# Autodesk Inventor assembly: Heatsink+fan RPi-5
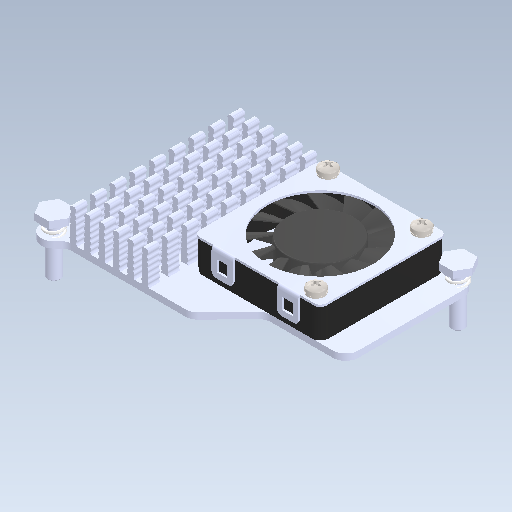
[picture p0: Inventor's stored thumbnail of the model, 512x512]
Saved by Autodesk Inventor 2021 (Build 250183000, 183)
## iProperties
Created: 2023-11-12
Part Number: Heatsink+fan RPi-5
Description: STEP AP214
Document SubType Name: Assembly
Designer: 22liatho
Sending System: SolidWorks 2021
Preprocessor: SwSTEP 2.0
Title: Heatsink+fan RPi-5.STEP
Revision Number: ANY
## Documents named in this file (7)
- C:\Users\22liatho\OneDrive - ABB Gymnasiet\Årskurs 3\Profil\Gymnasiearbete\GyArb Hållare CAD\CAD-filer\Raspberry_Pi_Heatsink+fan.iam
- C:\Users\22liatho\OneDrive - ABB Gymnasiet\Årskurs 3\Profil\Gymnasiearbete\GyArb Hållare CAD\CAD-filer\Heatsink-fan-base_RPi5.ipt
- C:\Users\22liatho\OneDrive - ABB Gymnasiet\Årskurs 3\Profil\Gymnasiearbete\GyArb Hållare CAD\CAD-filer\Fan_Assembly.iam
- C:\Users\22liatho\OneDrive - ABB Gymnasiet\Årskurs 3\Profil\Gymnasiearbete\GyArb Hållare CAD\CAD-filer\Fan_Cover.ipt
- C:\Users\22liatho\OneDrive - ABB Gymnasiet\Årskurs 3\Profil\Gymnasiearbete\GyArb Hållare CAD\CAD-filer\Spring-bolt_M2,5.iam
- C:\Users\22liatho\OneDrive - ABB Gymnasiet\Årskurs 3\Profil\Gymnasiearbete\GyArb Hållare CAD\CAD-filer\pan_head_cross_recess_screw_din_DIN_EN_ISO_7045_-_M2_x_10_-_Z_-_10N.ipt
- C:\Users\22liatho\OneDrive - ABB Gymnasiet\Årskurs 3\Profil\Gymnasiearbete\GyArb Hållare CAD\CAD-filer\plain_washer_small_grade_a_din_Washer_DIN_433_-_2.ipt
## Components (11 placed, 11 different names)
1. Heatsink-fan-base_RPi5_1 — Mate:1, Mate:2, Mate:3, Mate:4
2. final_assembly_2 [sub-assembly]
3. fan cover_3
4. Spring-bolt_M2,5_4 [sub-assembly] — Mate:1, Mate:2
5. Spring-bolt_M2,5_5 [sub-assembly] — Mate:3, Mate:4
6. pan head cross recess screw_din_DIN EN ISO 7045 - M2 x 10 - Z - 10N_6
7. pan head cross recess screw_din_DIN EN ISO 7045 - M2 x 10 - Z - 10N_7
8. pan head cross recess screw_din_DIN EN ISO 7045 - M2 x 10 - Z - 10N_8
9. plain washer small grade a_din_Washer DIN 433 - 2_9
10. plain washer small grade a_din_Washer DIN 433 - 2_10
11. plain washer small grade a_din_Washer DIN 433 - 2_11
## Relationships (4: Mate 4)
- Mate:1: Heatsink-fan-base_RPi5_1 ↔ Spring-bolt_M2,5_4
- Mate:2 (2.5 mm): Heatsink-fan-base_RPi5_1 ↔ Spring-bolt_M2,5_4
- Mate:3: Heatsink-fan-base_RPi5_1 ↔ Spring-bolt_M2,5_5
- Mate:4 (2.5 mm): Heatsink-fan-base_RPi5_1 ↔ Spring-bolt_M2,5_5
